# Autodesk Inventor assembly: Frame
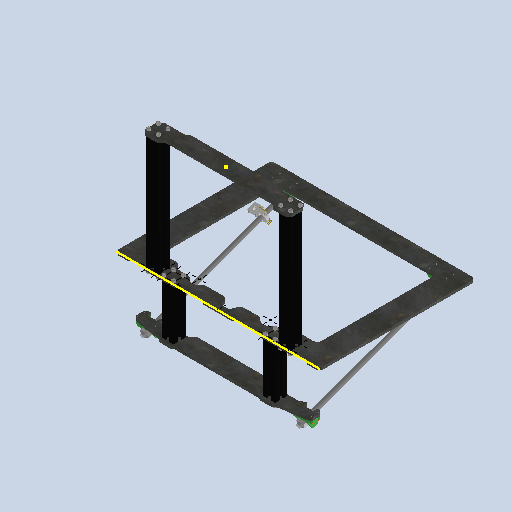
[picture p0: Inventor's stored thumbnail of the model, 512x512]
Saved by Autodesk Inventor 2023 (Build 270158000, 158)
## iProperties
Created: 2019-06-17
Part Number: Frame
Document SubType Name: Assembly
Designer: pepd9
Author: pepd9
## Documents named in this file (18)
- D:\000 - PEPCORP CLOUD\00- Legacy\Designs\MK3PRO P1\FRAME\Frame.iam
- D:\000 - PEPCORP CLOUD\00- Legacy\Designs\MK3PRO P1\FRAME\CENTER FRAME P1.2.ipt
- D:\000 - PEPCORP CLOUD\00- Legacy\Designs\MK3PRO P1\FRAME\FRONT PLATE P1.2.ipt
- D:\000 - PEPCORP CLOUD\00- Legacy\Designs\MK3PRO P1\FRAME\Long Extrusion.ipt
- D:\000 - PEPCORP CLOUD\00- Legacy\Designs\MK3PRO P1\COMPONENTS\90128A234_ZNC-PLTD ALLOY STL SCKT HEAD CAP SCREW.ipt
- D:\000 - PEPCORP CLOUD\00- Legacy\Designs\MK3PRO P1\FRAME\Short Extrusion.ipt
- D:\000 - PEPCORP CLOUD\00- Legacy\Designs\MK3PRO P1\FRAME\REAR PLATE P1.2.ipt
- D:\000 - PEPCORP CLOUD\00- Legacy\Designs\MK3PRO P1\FRAME\Angle Support Bottom Anchor.ipt
- D:\000 - PEPCORP CLOUD\00- Legacy\Designs\MK3PRO P1\FRAME\Angle Support Top Anchor.ipt
- D:\000 - PEPCORP CLOUD\00- Legacy\Designs\MK3PRO P1\COMPONENTS\WASHER_M10.ipt
- D:\000 - PEPCORP CLOUD\00- Legacy\Designs\MK3PRO P1\FRAME\Angle Support.ipt
- D:\000 - PEPCORP CLOUD\00- Legacy\Designs\MK3PRO P1\COMPONENTS\NUT_THIN_M10.ipt
- D:\000 - PEPCORP CLOUD\00- Legacy\Designs\MK3PRO P1\COMPONENTS\SHCS_M3_12.ipt
- D:\000 - PEPCORP CLOUD\00- Legacy\Designs\MK3PRO P1\COMPONENTS\M3 Nut.ipt
- D:\000 - PEPCORP CLOUD\00- Legacy\Designs\MK3PRO P1\COMPONENTS\SHCS_M3_18.ipt
- D:\000 - PEPCORP CLOUD\00- Legacy\Designs\MK3PRO P1\FRAME\Bed Cable Harness Rod Clamp.ipt
- D:\000 - PEPCORP CLOUD\00- Legacy\Designs\MK3PRO P1\FRAME\Bed Cable Harness.ipt
- D:\000 - PEPCORP CLOUD\00- Legacy\Designs\MK3PRO P1\FRAME\Bed Cable Harness Cable Clamp.ipt
## Components (96 placed, 17 different names)
1. CENTER FRAME P1.2:1 — Mate:1, Mate:2, Mate:3, Mate:4, Mate:5, Mate:6, Mate:7, Mate:8, Mate:9, Flush:1, Mate:23, Mate:24, Mate:25, Mate:28, Mate:37, Mate:38, Mate:39, Mate:40, Mate:41, Mate:42, Mate:43, Mate:44, Mate:45, Mate:46, Mate:47, Mate:48, Mate:49, Mate:50, Mate:51, Mate:52, Mate:53, Mate:54, Mate:55, Mate:56, Mate:57, Mate:58, Mate:59, Mate:60, Mate:61, Mate:62, Mate:63, Mate:64, Mate:65, Mate:66, Mate:96, Mate:97, Mate:98, Mate:99, Mate:100, Mate:101
2. FRONT PLATE P1.2:1 — Mate:12, Mate:13, Mate:14, Mate:15, Mate:16, Mate:17, Mate:18, Mate:19, Mate:20, Mate:21, Mate:22, Mate:26, Mate:27, Mate:29, Mate:30, Mate:31, Mate:32, Mate:33, Mate:34, Mate:35, Mate:36
3. Long Extrusion:1 — Mate:1, Mate:10, Mate:11, Mate:12, Mate:13, Mate:14
4. 90128A234_ZNC-PLTD ALLOY STL SCKT HEAD CAP SCREW:1 — Mate:2, Mate:3, Mate:10
5. 90128A234_ZNC-PLTD ALLOY STL SCKT HEAD CAP SCREW:2 — Mate:6, Mate:7
6. 90128A234_ZNC-PLTD ALLOY STL SCKT HEAD CAP SCREW:3 — Mate:5, Mate:8
7. 90128A234_ZNC-PLTD ALLOY STL SCKT HEAD CAP SCREW:4 — Mate:4, Mate:9, Mate:11
8. 90128A234_ZNC-PLTD ALLOY STL SCKT HEAD CAP SCREW:5 — Mate:15, Mate:19
9. 90128A234_ZNC-PLTD ALLOY STL SCKT HEAD CAP SCREW:6 — Mate:16, Mate:20
10. 90128A234_ZNC-PLTD ALLOY STL SCKT HEAD CAP SCREW:7 — Mate:17, Mate:22
11. 90128A234_ZNC-PLTD ALLOY STL SCKT HEAD CAP SCREW:8 — Mate:18, Mate:21
12. Long Extrusion:2 — Mate:25, Mate:26, Mate:27, Mate:28
13. 90128A234_ZNC-PLTD ALLOY STL SCKT HEAD CAP SCREW:9 — Mate:32, Mate:36
14. 90128A234_ZNC-PLTD ALLOY STL SCKT HEAD CAP SCREW:10 — Mate:31, Mate:35
15. 90128A234_ZNC-PLTD ALLOY STL SCKT HEAD CAP SCREW:11 — Mate:30, Mate:34
16. 90128A234_ZNC-PLTD ALLOY STL SCKT HEAD CAP SCREW:12 — Mate:29, Mate:33
17. 90128A234_ZNC-PLTD ALLOY STL SCKT HEAD CAP SCREW:13 — Mate:37, Mate:44
18. 90128A234_ZNC-PLTD ALLOY STL SCKT HEAD CAP SCREW:14 — Mate:38, Mate:42
19. 90128A234_ZNC-PLTD ALLOY STL SCKT HEAD CAP SCREW:15 — Mate:39, Mate:43
20. 90128A234_ZNC-PLTD ALLOY STL SCKT HEAD CAP SCREW:16 — Mate:40, Mate:41
21. Short Extrusion:1 — Mate:45, Mate:46, Mate:47
22. Short Extrusion:2 — Mate:48, Mate:49, Mate:50, Mate:67, Mate:68, Mate:69
23. 90128A234_ZNC-PLTD ALLOY STL SCKT HEAD CAP SCREW:17 — Mate:53, Mate:56
24. 90128A234_ZNC-PLTD ALLOY STL SCKT HEAD CAP SCREW:18 — Mate:54, Mate:58
25. 90128A234_ZNC-PLTD ALLOY STL SCKT HEAD CAP SCREW:19 — Mate:51, Mate:55
26. 90128A234_ZNC-PLTD ALLOY STL SCKT HEAD CAP SCREW:20 — Mate:52, Mate:57
27. 90128A234_ZNC-PLTD ALLOY STL SCKT HEAD CAP SCREW:21 — Mate:59, Mate:63
28. 90128A234_ZNC-PLTD ALLOY STL SCKT HEAD CAP SCREW:22 — Mate:60, Mate:64
29. 90128A234_ZNC-PLTD ALLOY STL SCKT HEAD CAP SCREW:23 — Mate:61, Mate:65
30. 90128A234_ZNC-PLTD ALLOY STL SCKT HEAD CAP SCREW:24 — Mate:62, Mate:66
31. REAR PLATE P1.2:1 — Mate:67, Mate:68, Mate:69, Mate:70, Mate:71, Mate:72, Mate:73, Mate:74, Mate:75, Mate:76, Mate:77, Mate:78, Mate:79, Mate:80, Mate:81, Mate:82, Mate:83, Mate:84, Mate:95, Mate:102, Mate:103
32. 90128A234_ZNC-PLTD ALLOY STL SCKT HEAD CAP SCREW:25 — Mate:70, Mate:83
33. 90128A234_ZNC-PLTD ALLOY STL SCKT HEAD CAP SCREW:26 — Mate:71, Mate:81
34. 90128A234_ZNC-PLTD ALLOY STL SCKT HEAD CAP SCREW:27 — Mate:73, Mate:84
35. 90128A234_ZNC-PLTD ALLOY STL SCKT HEAD CAP SCREW:28 — Mate:72, Mate:82
36. 90128A234_ZNC-PLTD ALLOY STL SCKT HEAD CAP SCREW:29 — Mate:76, Mate:78
37. 90128A234_ZNC-PLTD ALLOY STL SCKT HEAD CAP SCREW:30 — Mate:74, Mate:77
38. 90128A234_ZNC-PLTD ALLOY STL SCKT HEAD CAP SCREW:31 — Mate:75, Mate:79
39. 90128A234_ZNC-PLTD ALLOY STL SCKT HEAD CAP SCREW:32 — Mate:80, Mate:95
40. Angle Support Bottom Anchor:1 — Mate:102, Mate:104, Mate:106, Mate:107, Mate:108, Mate:109, Mate:168, Mate:169, Mate:170, Mate:171, Mate:172, Mate:173, Mate:174, Mate:175
41. Angle Support Bottom Anchor:2 — Mate:103, Mate:105, Mate:110, Mate:111, Mate:112, Mate:113, Mate:176, Mate:177, Mate:178, Mate:179, Mate:180, Mate:181, Mate:182, Mate:183
42. Angle Support Top Anchor:1 — Mate:96, Mate:98, Mate:99, Mate:104, Mate:114, Mate:115, Mate:116, Mate:117, Mate:122, Mate:156, Mate:157, Mate:158, Mate:159, Mate:184, Mate:185, Mate:186, Mate:187
43. Angle Support Top Anchor:2 — Mate:97, Mate:100, Mate:101, Mate:105, Mate:118, Mate:119, Mate:120, Mate:121, Mate:123, Mate:160, Mate:161, Mate:162, Mate:163, Mate:164, Mate:165, Mate:166, Mate:167
44. WASHER_M10:1 — Mate:116, Mate:117, Mate:138
45. WASHER_M10:2 — Mate:114, Mate:115, Mate:136
46. WASHER_M10:3 — Mate:119, Mate:120, Mate:130
47. WASHER_M10:4 — Mate:118, Mate:121, Mate:128
48. WASHER_M10:5 — Mate:110, Mate:111, Mate:149
49. WASHER_M10:6 — Mate:112, Mate:113, Mate:154
50. WASHER_M10:7 — Mate:106, Mate:107, Mate:141
51. WASHER_M10:8 — Mate:108, Mate:109, Mate:146
52. Angle Support:1 — Mate:122, Mate:132, Mate:133, Mate:134, Mate:135, Flush:2, Mate:140, Mate:142, Mate:144, Mate:145
53. Angle Support:2 — Mate:123, Mate:124, Mate:125, Mate:126, Mate:127, Flush:3, Mate:148, Mate:150, Mate:152, Mate:153, Mate:205, Mate:207
54. NUT_THIN_M10:1 — Mate:134, Mate:138, Mate:139
55. NUT_THIN_M10:2 — Mate:135, Mate:139
56. NUT_THIN_M10:3 — Mate:132, Mate:137, Flush:2
57. NUT_THIN_M10:4 — Mate:133, Mate:136, Mate:137
58. NUT_THIN_M10:5 — Mate:125, Mate:131, Flush:3
59. NUT_THIN_M10:6 — Mate:127, Mate:129, Mate:212
60. NUT_THIN_M10:7 — Mate:126, Mate:128, Mate:129
61. NUT_THIN_M10:8 — Mate:124, Mate:130, Mate:131
62. NUT_THIN_M10:9 — Mate:140, Mate:141, Mate:143
63. NUT_THIN_M10:10 — Mate:144, Mate:146, Mate:147
64. NUT_THIN_M10:11 — Mate:145, Mate:147
65. NUT_THIN_M10:12 — Mate:142, Mate:143
66. NUT_THIN_M10:13 — Mate:148, Mate:149, Mate:151
67. NUT_THIN_M10:14 — Mate:152, Mate:154, Mate:155
68. NUT_THIN_M10:15 — Mate:150, Mate:151
69. NUT_THIN_M10:16 — Mate:153, Mate:155, Flush:4
70. SHCS_M3_12:1 — Mate:171, Mate:175
71. SHCS_M3_12:2 — Mate:170, Mate:174
72. SHCS_M3_12:3 — Mate:169, Mate:172
73. SHCS_M3_12:4 — Mate:168, Mate:173
74. SHCS_M3_12:5 — Mate:179, Mate:180
75. SHCS_M3_12:6 — Mate:178, Mate:181
76. SHCS_M3_12:7 — Mate:177, Mate:183
77. SHCS_M3_12:8 — Mate:176, Mate:182
78. SHCS_M3_12:9 — Mate:156, Mate:184
79. SHCS_M3_12:10 — Mate:157, Mate:185
80. SHCS_M3_12:11 — Mate:158, Mate:186
81. SHCS_M3_12:12 — Mate:159, Mate:187
82. SHCS_M3_12:13 — Mate:163, Mate:167
83. SHCS_M3_12:14 — Mate:162, Mate:166
84. SHCS_M3_12:15 — Mate:161, Mate:165
85. SHCS_M3_12:16 — Mate:160, Mate:164
86. Bed Cable Harness Cable Clamp:2 — Mate:209, Mate:210, Mate:211, Mate:214, Mate:215, Mate:219, Mate:220
87. Bed Cable Harness Rod Clamp:2 — Mate:206, Mate:207, Mate:208, Mate:212, Mate:225, Angle:5, Mate:227, Angle:6
88. Bed Cable Harness:2 — Mate:205, Mate:206, Mate:208, Mate:209, Mate:210, Mate:211, Mate:213, Mate:216, Mate:217, Mate:218, Mate:221, Angle:3, Mate:223, Angle:4
89. M3 Nut:5 — Mate:221, Mate:222, Angle:3
90. M3 Nut:6 — Mate:223, Mate:224, Angle:4
91. M3 Nut:7 — Mate:225, Mate:226, Angle:5
92. M3 Nut:8 — Mate:227, Angle:6, Mate:228
93. SHCS_M3_18:5 — Mate:215, Mate:219, Mate:222
94. SHCS_M3_18:6 — Mate:216, Mate:218, Mate:228
95. SHCS_M3_18:7 — Mate:214, Mate:220, Mate:224
96. SHCS_M3_18:8 — Mate:213, Mate:217, Mate:226
## Relationships (209: Mate 201, Flush 4, Angle 4)
- Mate:1: CENTER FRAME P1.2:1 ↔ Long Extrusion:1
- Mate:2: CENTER FRAME P1.2:1 ↔ 90128A234_ZNC-PLTD ALLOY STL SCKT HEAD CAP SCREW:1
- Mate:3: CENTER FRAME P1.2:1 ↔ 90128A234_ZNC-PLTD ALLOY STL SCKT HEAD CAP SCREW:1
- Mate:4: CENTER FRAME P1.2:1 ↔ 90128A234_ZNC-PLTD ALLOY STL SCKT HEAD CAP SCREW:4
- Mate:5: CENTER FRAME P1.2:1 ↔ 90128A234_ZNC-PLTD ALLOY STL SCKT HEAD CAP SCREW:3
- Mate:6: CENTER FRAME P1.2:1 ↔ 90128A234_ZNC-PLTD ALLOY STL SCKT HEAD CAP SCREW:2
- Mate:7: CENTER FRAME P1.2:1 ↔ 90128A234_ZNC-PLTD ALLOY STL SCKT HEAD CAP SCREW:2
- Mate:8: CENTER FRAME P1.2:1 ↔ 90128A234_ZNC-PLTD ALLOY STL SCKT HEAD CAP SCREW:3
- Mate:9: CENTER FRAME P1.2:1 ↔ 90128A234_ZNC-PLTD ALLOY STL SCKT HEAD CAP SCREW:4
- Mate:10: Long Extrusion:1 ↔ 90128A234_ZNC-PLTD ALLOY STL SCKT HEAD CAP SCREW:1
- Mate:11: Long Extrusion:1 ↔ 90128A234_ZNC-PLTD ALLOY STL SCKT HEAD CAP SCREW:4
- Mate:12: FRONT PLATE P1.2:1 ↔ Long Extrusion:1
- Mate:13: FRONT PLATE P1.2:1 ↔ Long Extrusion:1
- Mate:14: FRONT PLATE P1.2:1 ↔ Long Extrusion:1
- Mate:15: FRONT PLATE P1.2:1 ↔ 90128A234_ZNC-PLTD ALLOY STL SCKT HEAD CAP SCREW:5
- Mate:16: FRONT PLATE P1.2:1 ↔ 90128A234_ZNC-PLTD ALLOY STL SCKT HEAD CAP SCREW:6
- Mate:17: FRONT PLATE P1.2:1 ↔ 90128A234_ZNC-PLTD ALLOY STL SCKT HEAD CAP SCREW:7
- Mate:18: FRONT PLATE P1.2:1 ↔ 90128A234_ZNC-PLTD ALLOY STL SCKT HEAD CAP SCREW:8
- Mate:19: FRONT PLATE P1.2:1 ↔ 90128A234_ZNC-PLTD ALLOY STL SCKT HEAD CAP SCREW:5
- Mate:20: FRONT PLATE P1.2:1 ↔ 90128A234_ZNC-PLTD ALLOY STL SCKT HEAD CAP SCREW:6
- Mate:21: FRONT PLATE P1.2:1 ↔ 90128A234_ZNC-PLTD ALLOY STL SCKT HEAD CAP SCREW:8
- Mate:22: FRONT PLATE P1.2:1 ↔ 90128A234_ZNC-PLTD ALLOY STL SCKT HEAD CAP SCREW:7
- Flush:1 (-245 mm): CENTER FRAME P1.2:1
- Mate:23: CENTER FRAME P1.2:1
- Mate:24 (-24.5 mm): CENTER FRAME P1.2:1
- Mate:25: CENTER FRAME P1.2:1 ↔ Long Extrusion:2
- Mate:26: FRONT PLATE P1.2:1 ↔ Long Extrusion:2
- Mate:27: FRONT PLATE P1.2:1 ↔ Long Extrusion:2
- Mate:28: CENTER FRAME P1.2:1 ↔ Long Extrusion:2
- Mate:29: FRONT PLATE P1.2:1 ↔ 90128A234_ZNC-PLTD ALLOY STL SCKT HEAD CAP SCREW:12
- Mate:30: FRONT PLATE P1.2:1 ↔ 90128A234_ZNC-PLTD ALLOY STL SCKT HEAD CAP SCREW:11
- Mate:31: FRONT PLATE P1.2:1 ↔ 90128A234_ZNC-PLTD ALLOY STL SCKT HEAD CAP SCREW:10
- Mate:32: FRONT PLATE P1.2:1 ↔ 90128A234_ZNC-PLTD ALLOY STL SCKT HEAD CAP SCREW:9
- Mate:33: FRONT PLATE P1.2:1 ↔ 90128A234_ZNC-PLTD ALLOY STL SCKT HEAD CAP SCREW:12
- Mate:34: FRONT PLATE P1.2:1 ↔ 90128A234_ZNC-PLTD ALLOY STL SCKT HEAD CAP SCREW:11
- Mate:35: FRONT PLATE P1.2:1 ↔ 90128A234_ZNC-PLTD ALLOY STL SCKT HEAD CAP SCREW:10
- Mate:36: FRONT PLATE P1.2:1 ↔ 90128A234_ZNC-PLTD ALLOY STL SCKT HEAD CAP SCREW:9
- Mate:37: CENTER FRAME P1.2:1 ↔ 90128A234_ZNC-PLTD ALLOY STL SCKT HEAD CAP SCREW:13
- Mate:38: CENTER FRAME P1.2:1 ↔ 90128A234_ZNC-PLTD ALLOY STL SCKT HEAD CAP SCREW:14
- Mate:39: CENTER FRAME P1.2:1 ↔ 90128A234_ZNC-PLTD ALLOY STL SCKT HEAD CAP SCREW:15
- Mate:40: CENTER FRAME P1.2:1 ↔ 90128A234_ZNC-PLTD ALLOY STL SCKT HEAD CAP SCREW:16
- Mate:41: CENTER FRAME P1.2:1 ↔ 90128A234_ZNC-PLTD ALLOY STL SCKT HEAD CAP SCREW:16
- Mate:42: CENTER FRAME P1.2:1 ↔ 90128A234_ZNC-PLTD ALLOY STL SCKT HEAD CAP SCREW:14
- Mate:43: CENTER FRAME P1.2:1 ↔ 90128A234_ZNC-PLTD ALLOY STL SCKT HEAD CAP SCREW:15
- Mate:44: CENTER FRAME P1.2:1 ↔ 90128A234_ZNC-PLTD ALLOY STL SCKT HEAD CAP SCREW:13
- Mate:45: CENTER FRAME P1.2:1 ↔ Short Extrusion:1
- Mate:46: CENTER FRAME P1.2:1 ↔ Short Extrusion:1
- Mate:47: CENTER FRAME P1.2:1 ↔ Short Extrusion:1
- Mate:48: CENTER FRAME P1.2:1 ↔ Short Extrusion:2
- Mate:49: CENTER FRAME P1.2:1 ↔ Short Extrusion:2
- Mate:50: CENTER FRAME P1.2:1 ↔ Short Extrusion:2
- Mate:51: CENTER FRAME P1.2:1 ↔ 90128A234_ZNC-PLTD ALLOY STL SCKT HEAD CAP SCREW:19
- Mate:52: CENTER FRAME P1.2:1 ↔ 90128A234_ZNC-PLTD ALLOY STL SCKT HEAD CAP SCREW:20
- Mate:53: CENTER FRAME P1.2:1 ↔ 90128A234_ZNC-PLTD ALLOY STL SCKT HEAD CAP SCREW:17
- Mate:54: CENTER FRAME P1.2:1 ↔ 90128A234_ZNC-PLTD ALLOY STL SCKT HEAD CAP SCREW:18
- Mate:55: CENTER FRAME P1.2:1 ↔ 90128A234_ZNC-PLTD ALLOY STL SCKT HEAD CAP SCREW:19
- Mate:56: CENTER FRAME P1.2:1 ↔ 90128A234_ZNC-PLTD ALLOY STL SCKT HEAD CAP SCREW:17
- Mate:57: CENTER FRAME P1.2:1 ↔ 90128A234_ZNC-PLTD ALLOY STL SCKT HEAD CAP SCREW:20
- Mate:58: CENTER FRAME P1.2:1 ↔ 90128A234_ZNC-PLTD ALLOY STL SCKT HEAD CAP SCREW:18
- Mate:59: CENTER FRAME P1.2:1 ↔ 90128A234_ZNC-PLTD ALLOY STL SCKT HEAD CAP SCREW:21
- Mate:60: CENTER FRAME P1.2:1 ↔ 90128A234_ZNC-PLTD ALLOY STL SCKT HEAD CAP SCREW:22
- Mate:61: CENTER FRAME P1.2:1 ↔ 90128A234_ZNC-PLTD ALLOY STL SCKT HEAD CAP SCREW:23
- Mate:62: CENTER FRAME P1.2:1 ↔ 90128A234_ZNC-PLTD ALLOY STL SCKT HEAD CAP SCREW:24
- Mate:63: CENTER FRAME P1.2:1 ↔ 90128A234_ZNC-PLTD ALLOY STL SCKT HEAD CAP SCREW:21
- Mate:64: CENTER FRAME P1.2:1 ↔ 90128A234_ZNC-PLTD ALLOY STL SCKT HEAD CAP SCREW:22
- Mate:65: CENTER FRAME P1.2:1 ↔ 90128A234_ZNC-PLTD ALLOY STL SCKT HEAD CAP SCREW:23
- Mate:66: CENTER FRAME P1.2:1 ↔ 90128A234_ZNC-PLTD ALLOY STL SCKT HEAD CAP SCREW:24
- Mate:67: Short Extrusion:2 ↔ REAR PLATE P1.2:1
- Mate:68: Short Extrusion:2 ↔ REAR PLATE P1.2:1
- Mate:69: Short Extrusion:2 ↔ REAR PLATE P1.2:1
- Mate:70: REAR PLATE P1.2:1 ↔ 90128A234_ZNC-PLTD ALLOY STL SCKT HEAD CAP SCREW:25
- Mate:71: REAR PLATE P1.2:1 ↔ 90128A234_ZNC-PLTD ALLOY STL SCKT HEAD CAP SCREW:26
- Mate:72: REAR PLATE P1.2:1 ↔ 90128A234_ZNC-PLTD ALLOY STL SCKT HEAD CAP SCREW:28
- Mate:73: REAR PLATE P1.2:1 ↔ 90128A234_ZNC-PLTD ALLOY STL SCKT HEAD CAP SCREW:27
- Mate:74: REAR PLATE P1.2:1 ↔ 90128A234_ZNC-PLTD ALLOY STL SCKT HEAD CAP SCREW:30
- Mate:75: REAR PLATE P1.2:1 ↔ 90128A234_ZNC-PLTD ALLOY STL SCKT HEAD CAP SCREW:31
- Mate:76: REAR PLATE P1.2:1 ↔ 90128A234_ZNC-PLTD ALLOY STL SCKT HEAD CAP SCREW:29
- Mate:77: REAR PLATE P1.2:1 ↔ 90128A234_ZNC-PLTD ALLOY STL SCKT HEAD CAP SCREW:30
- Mate:78: REAR PLATE P1.2:1 ↔ 90128A234_ZNC-PLTD ALLOY STL SCKT HEAD CAP SCREW:29
- Mate:79: REAR PLATE P1.2:1 ↔ 90128A234_ZNC-PLTD ALLOY STL SCKT HEAD CAP SCREW:31
- Mate:80: REAR PLATE P1.2:1 ↔ 90128A234_ZNC-PLTD ALLOY STL SCKT HEAD CAP SCREW:32
- Mate:81: REAR PLATE P1.2:1 ↔ 90128A234_ZNC-PLTD ALLOY STL SCKT HEAD CAP SCREW:26
- Mate:82: REAR PLATE P1.2:1 ↔ 90128A234_ZNC-PLTD ALLOY STL SCKT HEAD CAP SCREW:28
- Mate:83: REAR PLATE P1.2:1 ↔ 90128A234_ZNC-PLTD ALLOY STL SCKT HEAD CAP SCREW:25
- Mate:84: REAR PLATE P1.2:1 ↔ 90128A234_ZNC-PLTD ALLOY STL SCKT HEAD CAP SCREW:27
- Mate:95: REAR PLATE P1.2:1 ↔ 90128A234_ZNC-PLTD ALLOY STL SCKT HEAD CAP SCREW:32
- Mate:96: CENTER FRAME P1.2:1 ↔ Angle Support Top Anchor:1
- Mate:97: CENTER FRAME P1.2:1 ↔ Angle Support Top Anchor:2
- Mate:98: CENTER FRAME P1.2:1 ↔ Angle Support Top Anchor:1
- Mate:99: CENTER FRAME P1.2:1 ↔ Angle Support Top Anchor:1
- Mate:100: CENTER FRAME P1.2:1 ↔ Angle Support Top Anchor:2
- Mate:101: CENTER FRAME P1.2:1 ↔ Angle Support Top Anchor:2
- Mate:102: REAR PLATE P1.2:1 ↔ Angle Support Bottom Anchor:1
- Mate:103: REAR PLATE P1.2:1 ↔ Angle Support Bottom Anchor:2
- Mate:104: Angle Support Bottom Anchor:1 ↔ Angle Support Top Anchor:1
- Mate:105: Angle Support Bottom Anchor:2 ↔ Angle Support Top Anchor:2
- Mate:106: Angle Support Bottom Anchor:1 ↔ WASHER_M10:7
- Mate:107: Angle Support Bottom Anchor:1 ↔ WASHER_M10:7
- Mate:108: Angle Support Bottom Anchor:1 ↔ WASHER_M10:8
- Mate:109: Angle Support Bottom Anchor:1 ↔ WASHER_M10:8
- Mate:110: Angle Support Bottom Anchor:2 ↔ WASHER_M10:5
- Mate:111: Angle Support Bottom Anchor:2 ↔ WASHER_M10:5
- Mate:112: Angle Support Bottom Anchor:2 ↔ WASHER_M10:6
- Mate:113: Angle Support Bottom Anchor:2 ↔ WASHER_M10:6
- Mate:114: Angle Support Top Anchor:1 ↔ WASHER_M10:2
- Mate:115: Angle Support Top Anchor:1 ↔ WASHER_M10:2
- Mate:116: Angle Support Top Anchor:1 ↔ WASHER_M10:1
- Mate:117: Angle Support Top Anchor:1 ↔ WASHER_M10:1
- Mate:118: Angle Support Top Anchor:2 ↔ WASHER_M10:4
- Mate:119: Angle Support Top Anchor:2 ↔ WASHER_M10:3
- Mate:120: Angle Support Top Anchor:2 ↔ WASHER_M10:3
- Mate:121: Angle Support Top Anchor:2 ↔ WASHER_M10:4
- Mate:122: Angle Support Top Anchor:1 ↔ Angle Support:1
- Mate:123: Angle Support Top Anchor:2 ↔ Angle Support:2
- Mate:124: Angle Support:2 ↔ NUT_THIN_M10:8
- Mate:125: Angle Support:2 ↔ NUT_THIN_M10:5
- Mate:126: Angle Support:2 ↔ NUT_THIN_M10:7
- Mate:127: Angle Support:2 ↔ NUT_THIN_M10:6
- Mate:128: WASHER_M10:4 ↔ NUT_THIN_M10:7
- Mate:129: NUT_THIN_M10:6 ↔ NUT_THIN_M10:7
- Mate:130: WASHER_M10:3 ↔ NUT_THIN_M10:8
- Mate:131: NUT_THIN_M10:5 ↔ NUT_THIN_M10:8
- Mate:132: Angle Support:1 ↔ NUT_THIN_M10:3
- Mate:133: Angle Support:1 ↔ NUT_THIN_M10:4
- Mate:134: Angle Support:1 ↔ NUT_THIN_M10:1
- Mate:135: Angle Support:1 ↔ NUT_THIN_M10:2
- Mate:136: WASHER_M10:2 ↔ NUT_THIN_M10:4
- Mate:137: NUT_THIN_M10:3 ↔ NUT_THIN_M10:4
- Mate:138: WASHER_M10:1 ↔ NUT_THIN_M10:1
- Mate:139: NUT_THIN_M10:1 ↔ NUT_THIN_M10:2
- Flush:2 (5 mm): Angle Support:1 ↔ NUT_THIN_M10:3
- Flush:3 (5 mm): Angle Support:2 ↔ NUT_THIN_M10:5
- Mate:140: Angle Support:1 ↔ NUT_THIN_M10:9
- Mate:141: WASHER_M10:7 ↔ NUT_THIN_M10:9
- Mate:142: Angle Support:1 ↔ NUT_THIN_M10:12
- Mate:143: NUT_THIN_M10:9 ↔ NUT_THIN_M10:12
- Mate:144: Angle Support:1 ↔ NUT_THIN_M10:10
- Mate:145: Angle Support:1 ↔ NUT_THIN_M10:11
- Mate:146: WASHER_M10:8 ↔ NUT_THIN_M10:10
- Mate:147: NUT_THIN_M10:10 ↔ NUT_THIN_M10:11
- Mate:148: Angle Support:2 ↔ NUT_THIN_M10:13
- Mate:149: WASHER_M10:5 ↔ NUT_THIN_M10:13
- Mate:150: Angle Support:2 ↔ NUT_THIN_M10:15
- Mate:151: NUT_THIN_M10:13 ↔ NUT_THIN_M10:15
- Mate:152: Angle Support:2 ↔ NUT_THIN_M10:14
- Mate:153: Angle Support:2 ↔ NUT_THIN_M10:16
- Mate:154: WASHER_M10:6 ↔ NUT_THIN_M10:14
- Mate:155: NUT_THIN_M10:14 ↔ NUT_THIN_M10:16
- Mate:156: Angle Support Top Anchor:1 ↔ SHCS_M3_12:9
- Mate:157: Angle Support Top Anchor:1 ↔ SHCS_M3_12:10
- Mate:158: Angle Support Top Anchor:1 ↔ SHCS_M3_12:11
- Mate:159: Angle Support Top Anchor:1 ↔ SHCS_M3_12:12
- Mate:160: Angle Support Top Anchor:2 ↔ SHCS_M3_12:16
- Mate:161: Angle Support Top Anchor:2 ↔ SHCS_M3_12:15
- Mate:162: Angle Support Top Anchor:2 ↔ SHCS_M3_12:14
- Mate:163: Angle Support Top Anchor:2 ↔ SHCS_M3_12:13
- Mate:164: Angle Support Top Anchor:2 ↔ SHCS_M3_12:16
- Mate:165: Angle Support Top Anchor:2 ↔ SHCS_M3_12:15
- Mate:166: Angle Support Top Anchor:2 ↔ SHCS_M3_12:14
- Mate:167: Angle Support Top Anchor:2 ↔ SHCS_M3_12:13
- Mate:168: Angle Support Bottom Anchor:1 ↔ SHCS_M3_12:4
- Mate:169: Angle Support Bottom Anchor:1 ↔ SHCS_M3_12:3
- Mate:170: Angle Support Bottom Anchor:1 ↔ SHCS_M3_12:2
- Mate:171: Angle Support Bottom Anchor:1 ↔ SHCS_M3_12:1
- Mate:172: Angle Support Bottom Anchor:1 ↔ SHCS_M3_12:3
- Mate:173: Angle Support Bottom Anchor:1 ↔ SHCS_M3_12:4
- Mate:174: Angle Support Bottom Anchor:1 ↔ SHCS_M3_12:2
- Mate:175: Angle Support Bottom Anchor:1 ↔ SHCS_M3_12:1
- Mate:176: Angle Support Bottom Anchor:2 ↔ SHCS_M3_12:8
- Mate:177: Angle Support Bottom Anchor:2 ↔ SHCS_M3_12:7
- Mate:178: Angle Support Bottom Anchor:2 ↔ SHCS_M3_12:6
- Mate:179: Angle Support Bottom Anchor:2 ↔ SHCS_M3_12:5
- Mate:180: Angle Support Bottom Anchor:2 ↔ SHCS_M3_12:5
- Mate:181: Angle Support Bottom Anchor:2 ↔ SHCS_M3_12:6
- Mate:182: Angle Support Bottom Anchor:2 ↔ SHCS_M3_12:8
- Mate:183: Angle Support Bottom Anchor:2 ↔ SHCS_M3_12:7
- Mate:184: Angle Support Top Anchor:1 ↔ SHCS_M3_12:9
- Mate:185: Angle Support Top Anchor:1 ↔ SHCS_M3_12:10
- Mate:186: Angle Support Top Anchor:1 ↔ SHCS_M3_12:11
- Mate:187: Angle Support Top Anchor:1 ↔ SHCS_M3_12:12
- Flush:4 (40 mm): NUT_THIN_M10:16
- Mate:205: Angle Support:2 ↔ Bed Cable Harness:2
- Mate:206: Bed Cable Harness Rod Clamp:2 ↔ Bed Cable Harness:2
- Mate:207: Angle Support:2 ↔ Bed Cable Harness Rod Clamp:2
- Mate:208: Bed Cable Harness Rod Clamp:2 ↔ Bed Cable Harness:2
- Mate:209: Bed Cable Harness Cable Clamp:2 ↔ Bed Cable Harness:2
- Mate:210: Bed Cable Harness Cable Clamp:2 ↔ Bed Cable Harness:2
- Mate:211: Bed Cable Harness Cable Clamp:2 ↔ Bed Cable Harness:2
- Mate:212 (40 mm): NUT_THIN_M10:6 ↔ Bed Cable Harness Rod Clamp:2
- Mate:213: Bed Cable Harness:2 ↔ SHCS_M3_18:8
- Mate:214: Bed Cable Harness Cable Clamp:2 ↔ SHCS_M3_18:7
- Mate:215: Bed Cable Harness Cable Clamp:2 ↔ SHCS_M3_18:5
- Mate:216: Bed Cable Harness:2 ↔ SHCS_M3_18:6
- Mate:217: Bed Cable Harness:2 ↔ SHCS_M3_18:8
- Mate:218: Bed Cable Harness:2 ↔ SHCS_M3_18:6
- Mate:219: Bed Cable Harness Cable Clamp:2 ↔ SHCS_M3_18:5
- Mate:220: Bed Cable Harness Cable Clamp:2 ↔ SHCS_M3_18:7
- Mate:221: Bed Cable Harness:2 ↔ M3 Nut:5
- Mate:222: M3 Nut:5 ↔ SHCS_M3_18:5
- Angle:3 (0 deg): Bed Cable Harness:2 ↔ M3 Nut:5
- Mate:223: Bed Cable Harness:2 ↔ M3 Nut:6
- Mate:224: M3 Nut:6 ↔ SHCS_M3_18:7
- Angle:4 (0 deg): Bed Cable Harness:2 ↔ M3 Nut:6
- Mate:225: Bed Cable Harness Rod Clamp:2 ↔ M3 Nut:7
- Mate:226: M3 Nut:7 ↔ SHCS_M3_18:8
- Angle:5 (0 deg): Bed Cable Harness Rod Clamp:2 ↔ M3 Nut:7
- Mate:227: Bed Cable Harness Rod Clamp:2 ↔ M3 Nut:8
- Angle:6 (0 deg): Bed Cable Harness Rod Clamp:2 ↔ M3 Nut:8
- Mate:228: M3 Nut:8 ↔ SHCS_M3_18:6
